# Autodesk Inventor assembly: Main_assmebly_originalcat
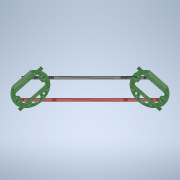
[picture p0: Inventor's stored thumbnail of the model, 180x180]
Saved by Autodesk Inventor 2022 (Build 260153000, 153)
## iProperties
Created: 2023-02-15
Part Number: Main_assmebly_originalcat
Document SubType Name: Assembly
Designer: scott
Author: scott
## Documents named in this file (4)
- C:\Users\scott\OneDrive\Documents\Cat project\Git_repository\Flinders_OpenCat\CAD components\Main_assmebly_originalcat.iam
- C:\Users\scott\OneDrive\Documents\Cat project\Git_repository\Flinders_OpenCat\CAD components\NybbleDIY\Imported Components\BellyPlate\BellyPlate.ipt
- C:\Users\scott\OneDrive\Documents\Cat project\Git_repository\Flinders_OpenCat\CAD components\Shoulder_assembly.iam
- C:\Users\scott\OneDrive\Documents\Cat project\Git_repository\Flinders_OpenCat\CAD components\NybbleDIY\Imported Components\Controller_Mount\Controller_Mount.ipt
## Components (5 placed, 3 different names)
1. BellyPlate:1 — Mate:1, Mate:2, Mate:3, Mate:4, Mate:5, Mate:6, Angle:1
2. Shoulder_assembly:1 [sub-assembly] — Mate:1, Mate:2, Mate:5, Mate:11
3. Shoulder_assembly:2 [sub-assembly] — Mate:3, Mate:4, Mate:6, Mate:7, Mate:8, Mate:9, Mate:10
4. Controller_Mount:1 — Mate:8, Mate:9, Flush:1
5. Controller_Mount:2 — Mate:7, Mate:10, Flush:1, Angle:1, Mate:11
## Relationships (13: Mate 11, Flush 1, Angle 1)
- Mate:1: BellyPlate:1 ↔ Shoulder_assembly:1
- Mate:2: BellyPlate:1 ↔ Shoulder_assembly:1
- Mate:3: BellyPlate:1 ↔ Shoulder_assembly:2
- Mate:4: BellyPlate:1 ↔ Shoulder_assembly:2
- Mate:5: BellyPlate:1 ↔ Shoulder_assembly:1
- Mate:6: BellyPlate:1 ↔ Shoulder_assembly:2
- Mate:7: Shoulder_assembly:2 ↔ Controller_Mount:2
- Mate:8: Shoulder_assembly:2 ↔ Controller_Mount:1
- Mate:9: Shoulder_assembly:2 ↔ Controller_Mount:1
- Mate:10: Shoulder_assembly:2 ↔ Controller_Mount:2
- Flush:1: Controller_Mount:1 ↔ Controller_Mount:2
- Angle:1 (90 deg): BellyPlate:1 ↔ Controller_Mount:2
- Mate:11: Shoulder_assembly:1 ↔ Controller_Mount:2
